# Autodesk Inventor assembly: Flex Holder V1
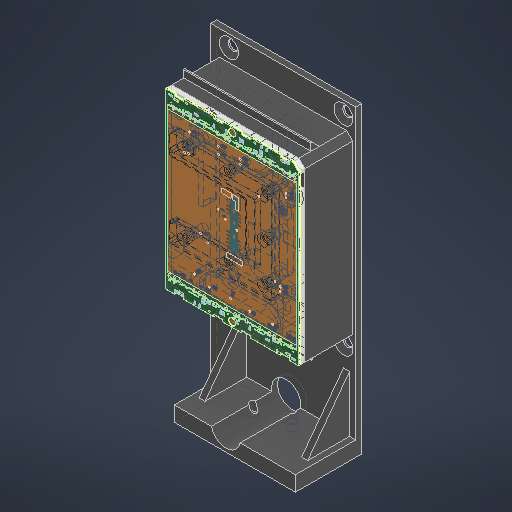
[picture p0: Inventor's stored thumbnail of the model, 512x512]
Saved by Autodesk Inventor 2027 (Build 310192060, 192F)
## iProperties
Created: 2025-07-01
Part Number: Flex Holder V1
Document SubType Name: Assembly
Designer: Caleb Fangmeier
Author: Caleb Fangmeier
## Documents named in this file (6)
- C:\Users\cfang\Desktop\nebraska-silicon-lab\Hardware\ETL\Module Assembly\FLEX Holder V2\Flex Holder V2.iam
- C:\Users\cfang\Desktop\nebraska-silicon-lab\Hardware\ETL\Module Assembly\FLEX Holder V2\Flex holder Base V2.ipt
- C:\Users\cfang\Desktop\nebraska-silicon-lab\Hardware\ETL\Module Assembly\Tamale Assembly Plate FLEX V1\Flex Cable Assembly V1.iam
- C:\Users\cfang\Desktop\nebraska-silicon-lab\Hardware\ETL\Module Assembly\FLEX Holder V2\Flex Circuit Clamp V2.ipt
- C:\Users\cfang\Desktop\nebraska-silicon-lab\Hardware\ETL\Module Assembly\FLEX Holder V2\Flex Holder Gasket V3.ipt
- C:\Users\cfang\Desktop\nebraska-silicon-lab\Hardware\ETL\modules\Tamale v1.6\ETL_ETROC_MODULE_v45_model\ETL_ETROC_MODULE_v45_model.iam
## Components (5 placed, 5 different names)
1. Flex Holder Gasket V3:1 — Flush:3, Flush:4, Mate:8, Mate:9, Flush:9, Flush:10
2. Flex holder Base V2:1 — Flush:3, Flush:4, Mate:3, Mate:5, Flush:7, Flush:8, Mate:6, Mate:7, Mate:8
3. Flex Cable Assembly V1:1 [sub-assembly] — Mate:3, Flush:7, Flush:8
4. Flex Circuit Clamp V2:1 — Mate:5, Mate:6, Mate:7
5. ETL_ETROC_MODULE_v45_model:1 [sub-assembly] — Mate:9, Flush:9, Flush:10
## Relationships (12: Flush 6, Mate 6)
- Flush:3: Flex Holder Gasket V3:1 ↔ Flex holder Base V2:1
- Flush:4: Flex Holder Gasket V3:1 ↔ Flex holder Base V2:1
- Mate:3 (0.35 mm): Flex holder Base V2:1 ↔ Flex Cable Assembly V1:1
- Mate:5: Flex holder Base V2:1 ↔ Flex Circuit Clamp V2:1
- Flush:7: Flex holder Base V2:1 ↔ Flex Cable Assembly V1:1
- Flush:8: Flex holder Base V2:1 ↔ Flex Cable Assembly V1:1
- Mate:6: Flex holder Base V2:1 ↔ Flex Circuit Clamp V2:1
- Mate:7 (0.1 mm): Flex holder Base V2:1 ↔ Flex Circuit Clamp V2:1
- Mate:8: Flex Holder Gasket V3:1 ↔ Flex holder Base V2:1
- Mate:9: Flex Holder Gasket V3:1 ↔ ETL_ETROC_MODULE_v45_model:1
- Flush:9: Flex Holder Gasket V3:1 ↔ ETL_ETROC_MODULE_v45_model:1
- Flush:10: Flex Holder Gasket V3:1 ↔ ETL_ETROC_MODULE_v45_model:1
